# Autodesk Inventor assembly: troys chassie
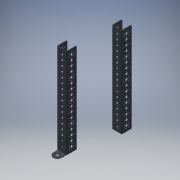
[picture p0: Inventor's stored thumbnail of the model, 180x180]
Saved by Autodesk Inventor 2016 (Build 200138000, 138)
## iProperties
Created: 2015-09-15
Part Number: troys chassie
Document SubType Name: Assembly
Designer: phi
Author: phi
## Documents named in this file (3)
- C:\Users\phi\Documents\GitHub\phi_robotics\3d-models\FTC_Tetrix_KOP_Block_Party\troys chassie.iam
- C:\Users\phi\Documents\GitHub\phi_robotics\3d-models\FTC_Tetrix_KOP_Block_Party\Tetrix_Kit_FTC\Autodesk Inventor Files\tetrix_c_channel-4.ipt
- C:\Users\phi\Documents\GitHub\phi_robotics\3d-models\FTC_Tetrix_KOP_Block_Party\Tetrix_Kit_FTC\Autodesk Inventor Files\tetrix_Lbracket-round.ipt
## Components (3 placed, 2 different names)
1. tetrix_c_channel-4:1 — Rigid:1
2. tetrix_c_channel-4:2
3. tetrix_Lbracket-round:1 — Rigid:1
## Relationships (1: WeldJoint 1)
- Rigid:1 [WeldJoint]: tetrix_c_channel-4:1 ↔ tetrix_Lbracket-round:1
